# Autodesk Inventor assembly: EnsambleRobot
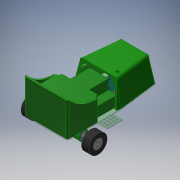
[picture p0: Inventor's stored thumbnail of the model, 180x180]
Saved by Autodesk Inventor 2017 (Build 210142000, 142)
## iProperties
Created: 2017-04-02
Part Number: EnsambleRobot
Document SubType Name: Assembly
Designer: Nick
Mass: 851.439 g
Surface Area: 3588.51 cm^2
Volume: 878.619 cm^3
Density: 0.969065 g/cm^3
Author: Nick
## Documents named in this file (9)
- C:\Users\Nick\Desktop\RobotCAD\EnsambleRobot.iam
- C:\Users\Nick\Desktop\RobotCAD\Base.ipt
- C:\Users\Nick\Desktop\RobotCAD\motor_w_wheel.iam
- C:\Users\Nick\Desktop\RobotCAD\front.ipt
- C:\Users\Nick\Documents\Inventor\Content Center Files\R2017\en-US\ANSI B18.2.2(06)\ANSI B18.2.2 - 5 - 44(06).ipt
- C:\Users\Nick\Desktop\RobotCAD\motor_holder.ipt
- C:\Users\Nick\Desktop\RobotCAD\rueda_loca.ipt
- C:\Users\Nick\Desktop\RobotCAD\Part29.ipt
- C:\Users\Nick\Desktop\RobotCAD\raspberrypi_b_+_(assembly).iam
## Components (11 placed, 8 different names)
1. Base:1 — Flush:1, Flush:2, Mate:3, Mate:4, Mate:5, Flush:5, Mate:6
2. motor_w_wheel:1 [sub-assembly] — Mate:1
3. motor_w_wheel:2 [sub-assembly] — Mate:2
4. front:1 — Flush:1, Flush:2
5. Hex Machine Screw Nut - Inch 5 - 44:1
6. Hex Machine Screw Nut - Inch 5 - 44:2
7. motor_holder:1 — Mate:2, Mate:3, Flush:3
8. motor_holder:2 — Mate:1, Mate:4, Flush:3
9. rueda_loca:2 — Mate:5
10. Back — Flush:5
11. raspberrypi_b_+_(assembly):1 [sub-assembly] — Mate:6
## Relationships (10: Mate 6, Flush 4)
- Flush:1: Base:1 ↔ front:1
- Flush:2 (70 mm): Base:1 ↔ front:1
- Mate:1: motor_w_wheel:1 ↔ motor_holder:2
- Mate:2: motor_w_wheel:2 ↔ motor_holder:1
- Mate:3: Base:1 ↔ motor_holder:1
- Mate:4: Base:1 ↔ motor_holder:2
- Flush:3: motor_holder:1 ↔ motor_holder:2
- Mate:5: Base:1 ↔ rueda_loca:2
- Flush:5: Base:1 ↔ Back
- Mate:6: Base:1 ↔ raspberrypi_b_+_(assembly):1
